# Autodesk Inventor assembly: wire nut with 2 wires
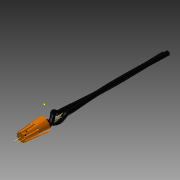
[picture p0: Inventor's stored thumbnail of the model, 180x180]
Saved by Autodesk Inventor 2014 (Build 180170000, 170)
## iProperties
Created: 2013-07-21
Part Number: wire nut with 2 wires
Document SubType Name: Assembly
Designer: Saville
Mass: 4.04289 g
Surface Area: 50.73 cm^2
Volume: 4.04289 cm^3
Density: 1 g/cm^3
Author: Saville
## Documents named in this file (3)
- C:\electrical nuts\terminal\wire nut with 2 wires.iam
- C:\electrical nuts\#18 orange.ipt
- C:\electrical nuts\terminal\Part4.ipt
## Components (2 placed, 2 different names)
1. #18 orange:1 — Flush:1, Flush:2, Mate:1, Flush:3
2. Part4:1 — Flush:1, Flush:2, Mate:1, Flush:3
## Relationships (4: Flush 3, Mate 1)
- Flush:1: #18 orange:1 ↔ Part4:1
- Flush:2 (36.5252 mm): #18 orange:1 ↔ Part4:1
- Mate:1: #18 orange:1 ↔ Part4:1
- Flush:3: #18 orange:1 ↔ Part4:1
